# Autodesk Inventor assembly: A2017_T3_01
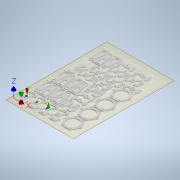
[picture p0: Inventor's stored thumbnail of the model, 180x180]
Saved by Autodesk Inventor 2020 (Build 240168000, 168)
## iProperties
Created: 2021-08-27
Part Number: A2017_T3_01
Document SubType Name: Assembly
Designer: Masato
Author: Masato
## Documents named in this file (7)
- C:\Inventor\SUSTAINA-OP_0311\Cam\A2017_T3_01.iam
- C:\Inventor\SUSTAINA-OP_0311\Cam\DisposableBoard.ipt
- C:\Inventor\SUSTAINA-OP_0311\LowerBody\Leg_joit\Leg_joint_roll_frame.ipt
- C:\Inventor\SUSTAINA-OP_0311\LowerBody\Leg_joit\Leg_joint_slider_frame.ipt
- C:\Inventor\SUSTAINA-OP_0311\LowerBody\Slider_crank\Slider_crank_horn.ipt
- C:\Inventor\SUSTAINA-OP_0311\LowerBody\Ankle\Ankle_front_frame.ipt
- C:\Inventor\SUSTAINA-OP_0311\UpperBody\Trunk\CrossRollerBearing\Outer_flange.ipt
## Components (37 placed, 6 different names)
1. DisposableBoard:1 — メイト:2, メイト:1, フラッシュ:1, フラッシュ:2, フラッシュ:12, 正接:1, フラッシュ:13, 角度:1, メイト:8, 正接:8, 角度:2, メイト:10, メイト:11, メイト:12, メイト:13, 角度:3, メイト:19, メイト:21, 角度:4, フラッシュ:15, メイト:22, メイト:23, メイト:24, メイト:25, メイト:26, メイト:27, メイト:28
2. Outer_flange:1 — フラッシュ:7
3. Leg_joint_roll_frame:6 — メイト:12, メイト:15, メイト:16, メイト:17, 正接:15, 正接:18
4. Leg_joint_roll_frame:7 — メイト:10, 正接:10, 正接:11, 角度:3, メイト:14, フラッシュ:14, メイト:15, メイト:18
5. Leg_joint_roll_frame:8 — メイト:13, メイト:14, フラッシュ:14, メイト:16, 正接:12
6. Leg_joint_roll_frame:9 — メイト:11, メイト:17, メイト:18, 正接:19, 正接:21
7. Ankle_front_frame:3 — メイト:21, 正接:13, 正接:14, 角度:4
8. Ankle_front_frame:4 — メイト:19, メイト:20, 正接:12
9. Leg_joint_slider_frame:9 — フラッシュ:15, メイト:22, 正接:15, メイト:29, 正接:16
10. Leg_joint_slider_frame:10 — メイト:23, メイト:29, 正接:16, メイト:30, 正接:17
11. Leg_joint_slider_frame:11 — メイト:24, メイト:30, 正接:17, 正接:20, メイト:32
12. Leg_joint_roll_frame:10 — メイト:25, メイト:31, 正接:21, 正接:23
13. Leg_joint_roll_frame:11 — メイト:26, 正接:18, 正接:19, 正接:20, メイト:31, 正接:22
14. Ankle_front_frame:5 — メイト:28, フラッシュ:16, 正接:23
15. Ankle_front_frame:6 — メイト:27, メイト:32, 正接:22, フラッシュ:16
16. Leg_joint_roll_frame:1 — フラッシュ:3, フラッシュ:4, フラッシュ:5, フラッシュ:10, フラッシュ:12, 正接:1, 正接:2, メイト:8
17. Leg_joint_roll_frame:3
18. Leg_joint_roll_frame:4
19. Leg_joint_roll_frame:5 — 正接:4, 正接:5, 正接:7
20. Leg_joint_slider_frame:1 — フラッシュ:6, フラッシュ:7, フラッシュ:13, 正接:2, メイト:5, 正接:3
21. Leg_joint_slider_frame:2 — フラッシュ:5, フラッシュ:6, メイト:5, 正接:3
22. Leg_joint_slider_frame:3 — メイト:20
23. Leg_joint_slider_frame:4
24. Leg_joint_slider_frame:5
25. Leg_joint_slider_frame:6 — メイト:7
26. Leg_joint_slider_frame:7
27. Leg_joint_slider_frame:8 — メイト:9
28. Outer_flange:2 — フラッシュ:9, 角度:1, 正接:7, 正接:8
29. Outer_flange:3
30. Outer_flange:4
31. Outer_flange:5 — 正接:13, 正接:14
32. Ankle_front_frame:1 — フラッシュ:10, 角度:2, 正接:9
33. Ankle_front_frame:2 — メイト:9
34. Slider_crank_horn:1 — フラッシュ:3, メイト:6, 正接:5
35. Slider_crank_horn:2 — フラッシュ:4, フラッシュ:9, メイト:6, 正接:4, メイト:7, 正接:9
36. Slider_crank_horn:3 — 正接:11
37. Slider_crank_horn:4 — 正接:10
## Component patterns: (4 elements, first: Leg_joint_roll_frame:1), (4 elements, first: Leg_joint_slider_frame:1 + Leg_joint_slider_frame:2), (4 elements, first: Outer_flange:2), (2 elements, first: Ankle_front_frame:1), (2 elements, first: Slider_crank_horn:1 + Slider_crank_horn:2)
## Relationships (70: Mate 30, Tangent 22, Flush 14, Angle 4)
- メイト:2 [Mate]: DisposableBoard:1
- メイト:1 [Mate]: DisposableBoard:1
- フラッシュ:1 [Flush]: DisposableBoard:1
- フラッシュ:2 [Flush]: DisposableBoard:1
- フラッシュ:3 [Flush]: Leg_joint_roll_frame:1 ↔ Slider_crank_horn:1
- フラッシュ:4 [Flush]: Leg_joint_roll_frame:1 ↔ Slider_crank_horn:2
- フラッシュ:5 [Flush]: Leg_joint_roll_frame:1 ↔ Leg_joint_slider_frame:2
- フラッシュ:6 [Flush]: Leg_joint_slider_frame:1 ↔ Leg_joint_slider_frame:2
- フラッシュ:7 [Flush]: Outer_flange:1 ↔ Leg_joint_slider_frame:1
- フラッシュ:9 [Flush]: Outer_flange:2 ↔ Slider_crank_horn:2
- フラッシュ:10 [Flush]: Leg_joint_roll_frame:1 ↔ Ankle_front_frame:1
- フラッシュ:12 [Flush] (2 mm): DisposableBoard:1 ↔ Leg_joint_roll_frame:1
- 正接:1 [Tangent] (2 mm): DisposableBoard:1 ↔ Leg_joint_roll_frame:1
- フラッシュ:13 [Flush] (2 mm): DisposableBoard:1 ↔ Leg_joint_slider_frame:1
- 正接:2 [Tangent] (2.5 mm): Leg_joint_roll_frame:1 ↔ Leg_joint_slider_frame:1
- メイト:5 [Mate] (2.5 mm): Leg_joint_slider_frame:1 ↔ Leg_joint_slider_frame:2
- 正接:3 [Tangent]: Leg_joint_slider_frame:1 ↔ Leg_joint_slider_frame:2
- メイト:6 [Mate] (2.5 mm): Slider_crank_horn:1 ↔ Slider_crank_horn:2
- 正接:4 [Tangent] (2.5 mm): Leg_joint_roll_frame:5 ↔ Slider_crank_horn:2
- 正接:5 [Tangent] (2.5 mm): Leg_joint_roll_frame:5 ↔ Slider_crank_horn:1
- メイト:7 [Mate] (2.5 mm): Leg_joint_slider_frame:6 ↔ Slider_crank_horn:2
- 角度:1 [Angle] (30 deg): DisposableBoard:1 ↔ Outer_flange:2
- メイト:8 [Mate]: DisposableBoard:1 ↔ Leg_joint_roll_frame:1
- 正接:7 [Tangent] (1 mm): Leg_joint_roll_frame:5 ↔ Outer_flange:2
- 正接:8 [Tangent] (2 mm): DisposableBoard:1 ↔ Outer_flange:2
- 角度:2 [Angle] (0 deg): DisposableBoard:1 ↔ Ankle_front_frame:1
- メイト:9 [Mate] (2.5 mm): Leg_joint_slider_frame:8 ↔ Ankle_front_frame:2
- 正接:9 [Tangent] (2.5 mm): Ankle_front_frame:1 ↔ Slider_crank_horn:2
- メイト:10 [Mate]: DisposableBoard:1 ↔ Leg_joint_roll_frame:7
- メイト:11 [Mate]: DisposableBoard:1 ↔ Leg_joint_roll_frame:9
- メイト:12 [Mate]: DisposableBoard:1 ↔ Leg_joint_roll_frame:6
- メイト:13 [Mate]: DisposableBoard:1 ↔ Leg_joint_roll_frame:8
- 正接:10 [Tangent] (2.5 mm): Leg_joint_roll_frame:7 ↔ Slider_crank_horn:4
- 正接:11 [Tangent] (2.5 mm): Leg_joint_roll_frame:7 ↔ Slider_crank_horn:3
- 角度:3 [Angle] (-90 deg): DisposableBoard:1 ↔ Leg_joint_roll_frame:7
- メイト:14 [Mate] (2.5 mm): Leg_joint_roll_frame:7 ↔ Leg_joint_roll_frame:8
- フラッシュ:14 [Flush]: Leg_joint_roll_frame:7 ↔ Leg_joint_roll_frame:8
- メイト:15 [Mate] (2.5 mm): Leg_joint_roll_frame:6 ↔ Leg_joint_roll_frame:7
- メイト:16 [Mate] (2.5 mm): Leg_joint_roll_frame:6 ↔ Leg_joint_roll_frame:8
- メイト:17 [Mate] (2.5 mm): Leg_joint_roll_frame:6 ↔ Leg_joint_roll_frame:9
- メイト:18 [Mate] (2.5 mm): Leg_joint_roll_frame:7 ↔ Leg_joint_roll_frame:9
- メイト:19 [Mate]: DisposableBoard:1 ↔ Ankle_front_frame:4
- メイト:20 [Mate] (2.5 mm): Ankle_front_frame:4 ↔ Leg_joint_slider_frame:3
- 正接:12 [Tangent] (2.5 mm): Leg_joint_roll_frame:8 ↔ Ankle_front_frame:4
- メイト:21 [Mate]: DisposableBoard:1 ↔ Ankle_front_frame:3
- 正接:13 [Tangent] (2.5 mm): Ankle_front_frame:3 ↔ Outer_flange:5
- 正接:14 [Tangent] (2.5 mm): Ankle_front_frame:3 ↔ Outer_flange:5
- 角度:4 [Angle] (180 deg): DisposableBoard:1 ↔ Ankle_front_frame:3
- フラッシュ:15 [Flush] (3 mm): DisposableBoard:1 ↔ Leg_joint_slider_frame:9
- メイト:22 [Mate]: DisposableBoard:1 ↔ Leg_joint_slider_frame:9
- メイト:23 [Mate]: DisposableBoard:1 ↔ Leg_joint_slider_frame:10
- メイト:24 [Mate]: DisposableBoard:1 ↔ Leg_joint_slider_frame:11
- メイト:25 [Mate]: DisposableBoard:1 ↔ Leg_joint_roll_frame:10
- メイト:26 [Mate]: DisposableBoard:1 ↔ Leg_joint_roll_frame:11
- メイト:27 [Mate]: DisposableBoard:1 ↔ Ankle_front_frame:6
- メイト:28 [Mate]: DisposableBoard:1 ↔ Ankle_front_frame:5
- 正接:15 [Tangent] (2.5 mm): Leg_joint_roll_frame:6 ↔ Leg_joint_slider_frame:9
- メイト:29 [Mate] (2.5 mm): Leg_joint_slider_frame:9 ↔ Leg_joint_slider_frame:10
- 正接:16 [Tangent]: Leg_joint_slider_frame:9 ↔ Leg_joint_slider_frame:10
- メイト:30 [Mate] (2.5 mm): Leg_joint_slider_frame:10 ↔ Leg_joint_slider_frame:11
- 正接:17 [Tangent]: Leg_joint_slider_frame:10 ↔ Leg_joint_slider_frame:11
- 正接:18 [Tangent] (2.5 mm): Leg_joint_roll_frame:6 ↔ Leg_joint_roll_frame:11
- 正接:19 [Tangent] (2.5 mm): Leg_joint_roll_frame:9 ↔ Leg_joint_roll_frame:11
- 正接:20 [Tangent] (2.5 mm): Leg_joint_slider_frame:11 ↔ Leg_joint_roll_frame:11
- メイト:31 [Mate] (2.5 mm): Leg_joint_roll_frame:10 ↔ Leg_joint_roll_frame:11
- 正接:21 [Tangent] (2.5 mm): Leg_joint_roll_frame:9 ↔ Leg_joint_roll_frame:10
- メイト:32 [Mate] (2.5 mm): Leg_joint_slider_frame:11 ↔ Ankle_front_frame:6
- 正接:22 [Tangent] (2.5 mm): Leg_joint_roll_frame:11 ↔ Ankle_front_frame:6
- フラッシュ:16 [Flush]: Ankle_front_frame:5 ↔ Ankle_front_frame:6
- 正接:23 [Tangent] (2.5 mm): Leg_joint_roll_frame:10 ↔ Ankle_front_frame:5
